# Autodesk Inventor assembly: Sun_ChairAssembly
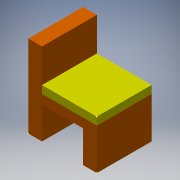
[picture p0: Inventor's stored thumbnail of the model, 180x180]
Saved by Autodesk Inventor 2016 (Build 200138000, 138)
## iProperties
Created: 2017-10-05
Part Number: Sun_ChairAssembly
Document SubType Name: Assembly
Designer: sun01147
Author: sun01147
## Documents named in this file (3)
- E:\IED7_SunT\IED7_Practice\IED7_Puzzle Cube\Sun_ChairAssembly.iam
- E:\IED7_SunT\IED7_Practice\IED7_Puzzle Cube\Sun_Base.ipt
- E:\IED7_SunT\IED7_Practice\IED7_Puzzle Cube\Sun_Cushion.ipt
## Components (2 placed, 2 different names)
1. Sun_Base:1 — Flush:1
2. Sun_Cushion:1 — Flush:1
## Relationships (1: Flush 1)
- Flush:1: Sun_Base:1 ↔ Sun_Cushion:1
